# Autodesk Inventor assembly: 811001-X1 & 811000 & 810501_Robot Shield & Quickstart & Shield Hardware Kit ASSY
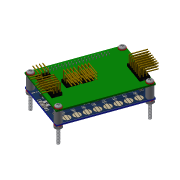
[picture p0: Inventor's stored thumbnail of the model, 180x180]
Saved by Autodesk Inventor 2015 (Build 190159000, 159)
## iProperties
Created: 2014-08-02
Part Number: 811001-X1 & 811000 & 810501_Robot Shield & Quickstart & Shield Hardware Kit ASSY
Document SubType Name: Assembly
Designer: david
Author: david
## Documents named in this file (7)
- C:\SharedDrive\Dropbox\FAST Robotics\Products\810001_FAST Robot Shield\CAD\810001_FAST Robot Shield\811001-X1 & 811000 & 810501_Robot Shield & Quickstart & Shield Hardware Kit ASSY.iam
- C:\SharedDrive\Dropbox\FAST Robotics\Products\810001_FAST Robot Shield\CAD\810001_FAST Robot Shield\810001-X1.iam
- C:\SharedDrive\Dropbox\FAST Robotics\Products\811000_Parallax Quickstart\CAD\811000_Parallax Quickstart\811000_Parallax Quickstart ASSY.iam
- C:\SharedDrive\Dropbox\FAST Robotics\Products\810501_Shield Hardware Kit\CAD\Imported Components\500505\500505.ipt
- C:\SharedDrive\Dropbox\FAST Robotics\Products\810501_Shield Hardware Kit\CAD\Imported Components\500506\500506.ipt
- C:\SharedDrive\Dropbox\FAST Robotics\Products\810501_Shield Hardware Kit\CAD\Imported Components\525000\525000.ipt
- C:\SharedDrive\Dropbox\FAST Robotics\Products\810501_Shield Hardware Kit\CAD\Imported Components\500507\500507.ipt
## Components (22 placed, 6 different names)
1. 810001-X1:1 [sub-assembly] — Mate:2, Angle:1, Insert:21, Insert:22, Insert:23, Insert:24
2. 811000_Parallax Quickstart ASSY:1 [sub-assembly] — Mate:2, Angle:1
3. 500505:2
4. 500506:3 — Insert:7, Insert:21
5. 500506:4 — Insert:8
6. 525000:2 — Insert:7, Insert:8
7. 500507:2
8. 500505:3
9. 500506:5 — Insert:23
10. 500506:6
11. 525000:3
12. 500507:3
13. 500505:4
14. 500506:7 — Insert:24
15. 500506:8
16. 525000:4
17. 500507:4
18. 500505:5
19. 500506:9 — Insert:22
20. 500506:10
21. 525000:5
22. 500507:5
## Relationships (26: Insert 20, Mate 5, Angle 1)
- Mate:2: 810001-X1:1 ↔ 811000_Parallax Quickstart ASSY:1
- Angle:1 (0 deg): 810001-X1:1 ↔ 811000_Parallax Quickstart ASSY:1
- [Mate]: 500506:3 ↔ 500506:4
- [Insert]: 500505:2 ↔ 500506:3
- [Insert]: 500506:4 ↔ 500507:2
- Insert:7 (1.524 mm): 500506:3 ↔ 525000:2
- Insert:8 (1.524 mm): 500506:4 ↔ 525000:2
- [Mate]: 500506:5 ↔ 500506:6
- [Insert]: 500505:3 ↔ 500506:5
- [Insert]: 500506:6 ↔ 500507:3
- [Insert] (1.524 mm): 500506:5 ↔ 525000:3
- [Insert] (1.524 mm): 500506:6 ↔ 525000:3
- [Mate]: 500506:7 ↔ 500506:8
- [Insert]: 500505:4 ↔ 500506:7
- [Insert]: 500506:8 ↔ 500507:4
- [Insert] (1.524 mm): 500506:7 ↔ 525000:4
- [Insert] (1.524 mm): 500506:8 ↔ 525000:4
- [Mate]: 500506:9 ↔ 500506:10
- [Insert]: 500505:5 ↔ 500506:9
- [Insert]: 500506:10 ↔ 500507:5
- [Insert] (1.524 mm): 500506:9 ↔ 525000:5
- [Insert] (1.524 mm): 500506:10 ↔ 525000:5
- Insert:21: 810001-X1:1 ↔ 500506:3
- Insert:22: 810001-X1:1 ↔ 500506:9
- Insert:23: 810001-X1:1 ↔ 500506:5
- Insert:24: 810001-X1:1 ↔ 500506:7
## Named parameters: d26_d20 = 0 mm, d27_d24 = 0 mm, d28_d25 = 0 mm, d31_d26_d20 = 0 mm, d32_d27_d24 = 0 mm, d33_d28_d25 = 0 mm, d34_d29 = 1.524 mm, d35_d30 = 1.524 mm, d36_d26_d20 = 0 mm, d37_d27_d24 = 0 mm, d38_d28_d25 = 0 mm, d39_d29 = 1.524 mm, d40_d30 = 1.524 mm, d41_d26_d20 = 0 mm, d42_d27_d24 = 0 mm, d43_d28_d25 = 0 mm, d44_d29 = 1.524 mm, d45_d30 = 1.524 mm
